# Autodesk Inventor assembly: Asiento - Ensamble
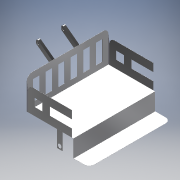
[picture p0: Inventor's stored thumbnail of the model, 180x180]
Saved by Autodesk Inventor 2019 (Build 230136000, 136)
## iProperties
Created: 2019-11-14
Part Number: Asiento - Ensamble
Document SubType Name: Weldment
Designer: eddysanoli
Weld Material: Welded Aluminum-6061
Mass: 369.022 g
Surface Area: 4964.76 cm^2
Volume: 136.673 cm^3
Density: 2.70004 g/cm^3
Author: eddysanoli
## Documents named in this file (4)
- E:\Archivos\Diseño\Inventor\Diseño Mecánico II\Proyecto - Hombre en Bicicleta\Mecanismos_Diseno\Asiento - Ensamble.iam
- E:\Archivos\Diseño\Inventor\Diseño Mecánico II\Proyecto - Hombre en Bicicleta\Mecanismos_Diseno\Asiento - Estructura Base.ipt
- E:\Archivos\Diseño\Inventor\Diseño Mecánico II\Proyecto - Hombre en Bicicleta\Mecanismos_Diseno\Asiento - Soporte Ruedas Delanteras.ipt
- E:\Archivos\Diseño\Inventor\Diseño Mecánico II\Proyecto - Hombre en Bicicleta\Mecanismos_Diseno\Asiento - Soporte Manija.ipt
## Components (5 placed, 3 different names)
1. Asiento - Estructura Base:1 — Coincidencia:2, Coincidencia:4, Coincidencia:5, Coincidencia:6, Nivelación:1, Nivelación:2, Coincidencia:7, Coincidencia:8, Nivelación:3, Nivelación:4, Tangente:1, Tangente:2
2. Asiento - Soporte Ruedas Delanteras:1 — Coincidencia:2, Coincidencia:4, Nivelación:2
3. Asiento - Soporte Ruedas Delanteras:2 — Coincidencia:5, Coincidencia:6, Nivelación:1
4. Asiento - Soporte Manija:1 — Coincidencia:8, Nivelación:3, Tangente:1
5. Asiento - Soporte Manija:2 — Coincidencia:7, Nivelación:4, Tangente:2
## Relationships (12: Mate 6, Flush 4, Tangent 2)
- Coincidencia:2 [Mate]: Asiento - Estructura Base:1 ↔ Asiento - Soporte Ruedas Delanteras:1
- Coincidencia:4 [Mate] (-25 mm): Asiento - Estructura Base:1 ↔ Asiento - Soporte Ruedas Delanteras:1
- Coincidencia:5 [Mate]: Asiento - Estructura Base:1 ↔ Asiento - Soporte Ruedas Delanteras:2
- Coincidencia:6 [Mate] (-25 mm): Asiento - Estructura Base:1 ↔ Asiento - Soporte Ruedas Delanteras:2
- Nivelación:1 [Flush] (120 mm): Asiento - Estructura Base:1 ↔ Asiento - Soporte Ruedas Delanteras:2
- Nivelación:2 [Flush] (120 mm): Asiento - Estructura Base:1 ↔ Asiento - Soporte Ruedas Delanteras:1
- Coincidencia:7 [Mate]: Asiento - Estructura Base:1 ↔ Asiento - Soporte Manija:2
- Coincidencia:8 [Mate]: Asiento - Estructura Base:1 ↔ Asiento - Soporte Manija:1
- Nivelación:3 [Flush] (-129 mm): Asiento - Estructura Base:1 ↔ Asiento - Soporte Manija:1
- Nivelación:4 [Flush] (-129 mm): Asiento - Estructura Base:1 ↔ Asiento - Soporte Manija:2
- Tangente:1 (-110 mm): Asiento - Estructura Base:1 ↔ Asiento - Soporte Manija:1
- Tangente:2 (110 mm): Asiento - Estructura Base:1 ↔ Asiento - Soporte Manija:2
